# Autodesk Inventor assembly: Lamp
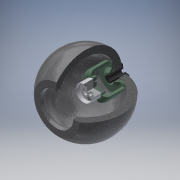
[picture p0: Inventor's stored thumbnail of the model, 180x180]
Saved by Autodesk Inventor 2018.2 (Build 222227000, 227)
## iProperties
Created: 2018-01-26
Part Number: Lamp
Material: Generisch
Document SubType Name: Assembly
Designer: JochenAlt
Author: JochenAlt
## Documents named in this file (8)
- D:\Projects\concretelamp\CAD\Lamp.iam
- D:\Projects\concretelamp\CAD\CableStrainRelief.ipt
- D:\Projects\concretelamp\CAD\Inlet.ipt
- D:\Projects\concretelamp\CAD\Lamp.ipt
- D:\Projects\concretelamp\CAD\Bulb GU10\Bulb GU10.iam
- D:\Projects\concretelamp\CAD\GU10-Socket.ipt
- C:\Users\JochenAlt\Documents\Inventor\Content Center Files\R2018\de-DE\DIN 912\DIN 912 - M3 x 0,5 x 12 x 10,75.ipt
- C:\Users\JochenAlt\Documents\Inventor\Content Center Files\R2018\de-DE\AS 1112 (2)\AS 1112 - M3  Typ 8.ipt
## Components (9 placed, 7 different names)
1. Kabelzugentlastung:1 — Passend:3, Passend:21, Passend:22, Passend:23
2. V5 Inlet:1 — Passend:22, Passend:23, Passend:24, Passend:25, Passend:26, Passend:29, Passend:35, Passend:37
3. Lamp:1 — Passend:3, Passend:21
4. Bulb GU10:1 [sub-assembly] — Passend:19, Passend:24, Passend:27, Passend:28
5. GU10-Socket:1 — Passend:19, Passend:25, Passend:26, Passend:27, Passend:28, Passend:29, Passend:30, Passend:31, Passend:32, Passend:33
6. DIN 912 - ersetzt durch DIN EN ISO 4762 M3 x 12:1 — Passend:30, Passend:31, Passend:34
7. DIN 912 - ersetzt durch DIN EN ISO 4762 M3 x 12:2 — Passend:32, Passend:33, Passend:36
8. AS 1112 (2) - Metrisch M3  Typ 8:1 — Passend:34, Passend:35
9. AS 1112 (2) - Metrisch M3  Typ 8:2 — Passend:36, Passend:37
## Relationships (19: Mate 19)
- Passend:3 [Mate]: Kabelzugentlastung:1 ↔ Lamp:1
- Passend:19 [Mate]: Bulb GU10:1 ↔ GU10-Socket:1
- Passend:21 [Mate]: Kabelzugentlastung:1 ↔ Lamp:1
- Passend:22 [Mate]: Kabelzugentlastung:1 ↔ V5 Inlet:1
- Passend:23 [Mate] (-2.8 mm): Kabelzugentlastung:1 ↔ V5 Inlet:1
- Passend:24 [Mate]: V5 Inlet:1 ↔ Bulb GU10:1
- Passend:25 [Mate]: V5 Inlet:1 ↔ GU10-Socket:1
- Passend:26 [Mate] (0.3 mm): V5 Inlet:1 ↔ GU10-Socket:1
- Passend:27 [Mate]: Bulb GU10:1 ↔ GU10-Socket:1
- Passend:28 [Mate] (0.3 mm): Bulb GU10:1 ↔ GU10-Socket:1
- Passend:29 [Mate]: V5 Inlet:1 ↔ GU10-Socket:1
- Passend:30 [Mate]: GU10-Socket:1 ↔ DIN 912 - ersetzt durch DIN EN ISO 4762 M3 x 12:1
- Passend:31 [Mate]: GU10-Socket:1 ↔ DIN 912 - ersetzt durch DIN EN ISO 4762 M3 x 12:1
- Passend:32 [Mate]: GU10-Socket:1 ↔ DIN 912 - ersetzt durch DIN EN ISO 4762 M3 x 12:2
- Passend:33 [Mate]: GU10-Socket:1 ↔ DIN 912 - ersetzt durch DIN EN ISO 4762 M3 x 12:2
- Passend:34 [Mate]: DIN 912 - ersetzt durch DIN EN ISO 4762 M3 x 12:1 ↔ AS 1112 (2) - Metrisch M3  Typ 8:1
- Passend:35 [Mate]: V5 Inlet:1 ↔ AS 1112 (2) - Metrisch M3  Typ 8:1
- Passend:36 [Mate]: DIN 912 - ersetzt durch DIN EN ISO 4762 M3 x 12:2 ↔ AS 1112 (2) - Metrisch M3  Typ 8:2
- Passend:37 [Mate]: V5 Inlet:1 ↔ AS 1112 (2) - Metrisch M3  Typ 8:2
